# Autodesk Inventor assembly: transmission
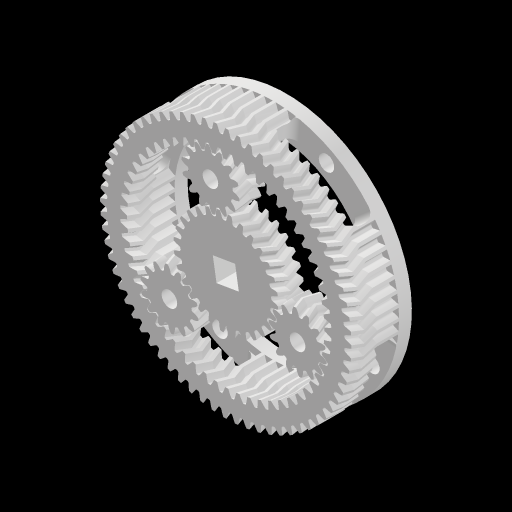
[picture p0: Inventor's stored thumbnail of the model, 512x512]
Saved by Autodesk Inventor 2024.1 (Build 281209000, 209)
## iProperties
Created: 2025-05-13
Part Number: transmission
Document SubType Name: Assembly
Designer: Teddy
Author: Teddy
## Documents named in this file (4)
- C:\Users\Teddy\OneDrive\Desktop\VEX-CAD-Inventor-1.4.0\pushBack\PushBackBot2\transmission.iam
- C:\Users\Teddy\OneDrive\Desktop\VEX-CAD-Inventor-1.4.0\pushBack\PushBackBot2\HerringBoneRingGear.ipt
- C:\Users\Teddy\OneDrive\Desktop\VEX-CAD-Inventor-1.4.0\pushBack\PushBackBot2\HerringBoneSunGear.ipt
- C:\Users\Teddy\OneDrive\Desktop\VEX-CAD-Inventor-1.4.0\pushBack\PushBackBot2\HerringBonePlanetGear.ipt
## Components (5 placed, 3 different names)
1. HerringBoneRingGear:1 — Insert:1
2. HerringBoneSunGear:1 — Insert:1
3. HerringBonePlanetGear:1
4. HerringBonePlanetGear:2
5. HerringBonePlanetGear:3
## Relationships (1: Insert 1)
- Insert:1: HerringBoneRingGear:1 ↔ HerringBoneSunGear:1
